# Autodesk Inventor assembly: PrinterMini
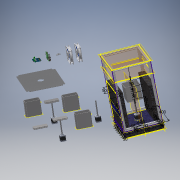
[picture p0: Inventor's stored thumbnail of the model, 180x180]
Saved by Autodesk Inventor 2016 (Build 200138000, 138)
## iProperties
Created: 2015-08-01
Part Number: PrinterMini
Document SubType Name: Assembly
Designer: myhome
Author: myhome
## Documents named in this file (14)
- C:\Users\myhome\Documents\Inventor\Printer\PrinterMini.iam
- C:\Users\myhome\Documents\Inventor\Printer\EpoxyGraniteBase\BaseMini.iam
- C:\Users\myhome\Documents\Inventor\Printer\FrameExtruded\FrameMini.iam
- C:\Users\myhome\Documents\Inventor\Printer\PistonFrame\PistonFeederFrameMini.iam
- C:\Users\myhome\Documents\Inventor\Printer\PistonFrame\PistonWorkFrameMini.iam
- C:\Users\myhome\Documents\Inventor\Printer\Nema17Motor\Nema17Stepper.iam
- C:\Users\myhome\Documents\Inventor\Printer\LinearActuator\LinearActuatorMini.iam
- C:\Users\myhome\Documents\Inventor\Printer\PistonHead\PistonFeederHeadMini.iam
- C:\Users\myhome\Documents\Inventor\Printer\FrameSheetMetal\FrameSheetLaserViewportMini.ipt
- C:\Users\myhome\Documents\Inventor\Printer\PistonHead\PistonWorkHeadMini.iam
- C:\Users\myhome\Documents\Inventor\Printer\SilverstoneFan\SilverstoneFQ121.iam
- C:\Users\myhome\Documents\Inventor\Printer\RaspberryPiCamera\RaspberryPiCamera.ipt
- C:\Users\myhome\Documents\Inventor\Printer\RaspberryPi2\RaspberryPi2.iam
- C:\Users\myhome\Documents\Inventor\Printer\GShield\GShield.iam
## Components (24 placed, 13 different names)
1. BaseMini:1 [sub-assembly] — Rigid:1, Rigid:5
2. FrameMini:1 [sub-assembly] — Rigid:1
3. PistonFrameMini:1 [sub-assembly]
4. PistonFrameMini:2 [sub-assembly]
5. PistonWorkFrameMini:1 [sub-assembly] — Rigid:9
6. Nema17Stepper:1 [sub-assembly] — Rigid:5, Rotational:1
7. LinearActuatorMini:1 [sub-assembly] — Rigid:7, Rotational:2
8. LinearActuatorMini:2 [sub-assembly] — Rigid:6, Rotational:3
9. LinearActuatorMini:3 [sub-assembly] — Rotational:1, Rigid:8, Rigid:9
10. PistonFeederHeadMini:3 [sub-assembly] — Rigid:7
11. PistonFeederHeadMini:4 [sub-assembly] — Rigid:6
12. FrameSheetLaserViewportMini:1
13. PistonWorkHeadMini:1 [sub-assembly] — Rigid:8
14. Nema17Stepper:2 [sub-assembly] — Rotational:2
15. Nema17Stepper:3 [sub-assembly] — Rotational:3
16. SilverstoneFQ121:2 [sub-assembly]
17. SilverstoneFQ121:3 [sub-assembly]
18. RaspberryPiCamera:1
19. RaspberryPi2:1 [sub-assembly]
20. GShield:1 [sub-assembly]
21. PistonFrameMini:3 [sub-assembly]
22. PistonFeederHeadMini:5 [sub-assembly]
23. LinearActuatorMini:5 [sub-assembly] — Rotational:4
24. Nema17Stepper:6 [sub-assembly] — Rotational:4
## Relationships (10: WeldJoint 6, RevoluteJoint 4)
- Rigid:1 [WeldJoint]: BaseMini:1 ↔ FrameMini:1
- Rigid:5 [WeldJoint]: BaseMini:1 ↔ Nema17Stepper:1
- Rotational:1 [RevoluteJoint]: Nema17Stepper:1 ↔ LinearActuatorMini:3
- Rigid:6 [WeldJoint]: LinearActuatorMini:2 ↔ PistonFeederHeadMini:4
- Rigid:7 [WeldJoint]: LinearActuatorMini:1 ↔ PistonFeederHeadMini:3
- Rigid:8 [WeldJoint]: LinearActuatorMini:3 ↔ PistonWorkHeadMini:1
- Rigid:9 [WeldJoint]: PistonWorkFrameMini:1 ↔ LinearActuatorMini:3
- Rotational:2 [RevoluteJoint]: LinearActuatorMini:1 ↔ Nema17Stepper:2
- Rotational:3 [RevoluteJoint]: LinearActuatorMini:2 ↔ Nema17Stepper:3
- Rotational:4 [RevoluteJoint]: LinearActuatorMini:5 ↔ Nema17Stepper:6
